# Autodesk Inventor assembly: Assembly1
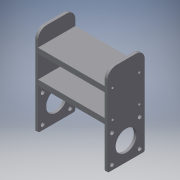
[picture p0: Inventor's stored thumbnail of the model, 180x180]
Saved by Autodesk Inventor 2016 SP1 (Build 200210100, 210)
## iProperties
Created: 2018-04-30
Part Number: Assembly1
Material: 一般
Document SubType Name: Assembly
Designer: kobay
Author: kobay
## Documents named in this file (3)
- C:\Users\kobay\Documents\Inventor\lancer_test_robot\Assembly1.iam
- C:\Users\kobay\Documents\Inventor\lancer_test_robot\body1.ipt
- C:\Users\kobay\Documents\Inventor\lancer_test_robot\body2.ipt
## Components (4 placed, 2 different names)
1. body1:1 — メイト:4, メイト:5, メイト:6, メイト:9
2. body1:2 — メイト:1, メイト:2, メイト:3, メイト:7, メイト:8
3. body2:1 — メイト:1, メイト:2, メイト:3, メイト:4, メイト:5, メイト:6
4. body2:2 — メイト:7, メイト:8, メイト:9
## Relationships (9: Mate 9)
- メイト:1 [Mate]: body1:2 ↔ body2:1
- メイト:2 [Mate]: body1:2 ↔ body2:1
- メイト:3 [Mate]: body1:2 ↔ body2:1
- メイト:4 [Mate]: body1:1 ↔ body2:1
- メイト:5 [Mate]: body1:1 ↔ body2:1
- メイト:6 [Mate]: body1:1 ↔ body2:1
- メイト:7 [Mate]: body1:2 ↔ body2:2
- メイト:8 [Mate]: body1:2 ↔ body2:2
- メイト:9 [Mate]: body1:1 ↔ body2:2
